# Autodesk Inventor assembly: Assembly2
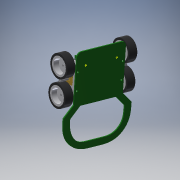
[picture p0: Inventor's stored thumbnail of the model, 180x180]
Saved by Autodesk Inventor 2016 (Build 200138000, 138)
## iProperties
Created: 2017-05-26
Part Number: Assembly2
Material: Ogólny
Document SubType Name: Assembly
Designer: Karol
Author: Karol
## Documents named in this file (12)
- D:\Git\MicromouseDixi\hardware\models\Dixi.iam
- D:\Git\MicromouseDixi\hardware\models\wheel.ipt
- D:\Git\MicromouseDixi\hardware\models\togh.ipt
- D:\Git\MicromouseDixi\hardware\models\bolt.ipt
- D:\Git\MicromouseDixi\hardware\models\magnet.ipt
- D:\Git\MicromouseDixi\hardware\models\mainpcb.ipt
- D:\Git\MicromouseDixi\hardware\models\motor.ipt
- D:\ele\MicroMouse\v2\hardware\models\top_mount.ipt
- D:\Git\MicromouseDixi\hardware\models\XSM_0203_03_1.ipt
- D:\Git\MicromouseDixi\hardware\models\XFM_020406_03_233.ipt
- D:\Git\MicromouseDixi\hardware\models\enc_pcb.ipt
- D:\Git\MicromouseDixi\hardware\models\tyre.ipt
## Components (31 placed, 11 different names)
1. mainpcb:1 — Rotational:1, Rigid:47, Rigid:48, Rigid:64, Rigid:65
2. bolt:3 — Rigid:15, Rigid:45
3. bolt:4 — Rigid:14, Rigid:46
4. wheel:3 — Rigid:15, Rigid:50
5. wheel:4 — Rigid:14, Rigid:49
6. magnet:4
7. togh:2 — Rigid:39, Rigid:40, Rigid:41, Rigid:44, Rotational:1, Rigid:47
8. motor:1 — Rigid:39
9. top_mount:1 — Rigid:40
10. XSM_0203_03_1:1 — Rigid:42, Rigid:45
11. XFM_020406_03_233:1 — Rigid:41, Rigid:42
12. XSM_0203_03_1:2 — Rigid:46
13. XFM_020406_03_233:2 — Rigid:44
14. enc_pcb:1 — Rigid:48
15. tyre:1 — Rigid:49
16. tyre:2 — Rigid:50
17. bolt:5 — Rigid:51, Rigid:56
18. bolt:6 — Rigid:52, Rigid:53, Rigid:59
19. wheel:5 — Rigid:51, Rigid:63
20. wheel:6 — Rigid:52, Rigid:62
21. magnet:5 — Rigid:53
22. togh:3 — Rigid:54, Rigid:55, Rigid:58, Rigid:60, Rigid:64
23. motor:2 — Rigid:54
24. top_mount:2 — Rigid:55
25. XSM_0203_03_1:3 — Rigid:56, Rigid:57
26. XFM_020406_03_233:3 — Rigid:57, Rigid:58
27. XSM_0203_03_1:4 — Rigid:59, Rigid:61
28. XFM_020406_03_233:4 — Rigid:60, Rigid:61
29. enc_pcb:2 — Rigid:65
30. tyre:3 — Rigid:62
31. tyre:4 — Rigid:63
## Relationships (31: WeldJoint 30, RevoluteJoint 1)
- Rigid:14 [WeldJoint] (-1.8 mm): bolt:4 ↔ wheel:4
- Rigid:15 [WeldJoint] (-1.8 mm): bolt:3 ↔ wheel:3
- [WeldJoint]: bolt:4 ↔ magnet:4
- Rigid:39 [WeldJoint]: togh:2 ↔ motor:1
- Rigid:40 [WeldJoint]: togh:2 ↔ top_mount:1
- Rigid:41 [WeldJoint] (-1.5 mm): togh:2 ↔ XFM_020406_03_233:1
- Rigid:42 [WeldJoint]: XSM_0203_03_1:1 ↔ XFM_020406_03_233:1
- [WeldJoint]: XSM_0203_03_1:2 ↔ XFM_020406_03_233:2
- Rigid:44 [WeldJoint] (1 mm): togh:2 ↔ XFM_020406_03_233:2
- Rigid:45 [WeldJoint]: bolt:3 ↔ XSM_0203_03_1:1
- Rigid:46 [WeldJoint]: bolt:4 ↔ XSM_0203_03_1:2
- Rotational:1 [RevoluteJoint]: mainpcb:1 ↔ togh:2
- Rigid:47 [WeldJoint]: mainpcb:1 ↔ togh:2
- Rigid:48 [WeldJoint]: mainpcb:1 ↔ enc_pcb:1
- Rigid:49 [WeldJoint]: wheel:4 ↔ tyre:1
- Rigid:50 [WeldJoint]: wheel:3 ↔ tyre:2
- Rigid:51 [WeldJoint] (-1.8 mm): bolt:5 ↔ wheel:5
- Rigid:52 [WeldJoint] (-1.8 mm): bolt:6 ↔ wheel:6
- Rigid:53 [WeldJoint]: bolt:6 ↔ magnet:5
- Rigid:54 [WeldJoint]: togh:3 ↔ motor:2
- Rigid:55 [WeldJoint]: togh:3 ↔ top_mount:2
- Rigid:56 [WeldJoint]: bolt:5 ↔ XSM_0203_03_1:3
- Rigid:57 [WeldJoint]: XSM_0203_03_1:3 ↔ XFM_020406_03_233:3
- Rigid:58 [WeldJoint] (-1.5 mm): togh:3 ↔ XFM_020406_03_233:3
- Rigid:59 [WeldJoint]: bolt:6 ↔ XSM_0203_03_1:4
- Rigid:60 [WeldJoint] (1 mm): togh:3 ↔ XFM_020406_03_233:4
- Rigid:61 [WeldJoint]: XSM_0203_03_1:4 ↔ XFM_020406_03_233:4
- Rigid:62 [WeldJoint]: wheel:6 ↔ tyre:3
- Rigid:63 [WeldJoint]: wheel:5 ↔ tyre:4
- Rigid:64 [WeldJoint]: mainpcb:1 ↔ togh:3
- Rigid:65 [WeldJoint]: mainpcb:1 ↔ enc_pcb:2
## Named parameters: d111_d4 = -1.8 mm, d112_d5 = 0.127925 deg, d113_d6 = -1.8 mm, d114_d7 = -6.839272 deg, d117_d14 = 0 mm, d118_d15 = 2.56641 deg, d234_d233 = 0 mm
